# Autodesk Inventor assembly: Ensamble EVA
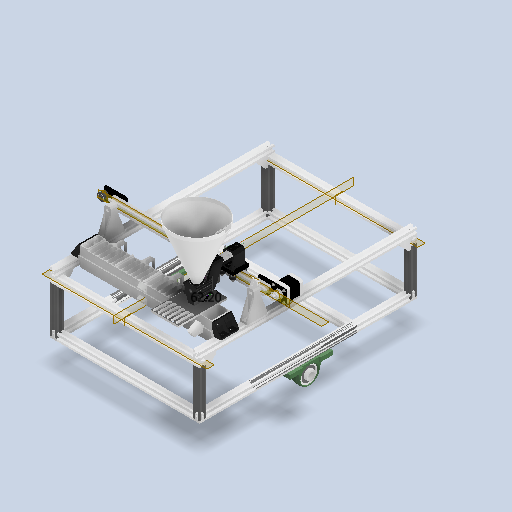
[picture p0: Inventor's stored thumbnail of the model, 512x512]
Saved by Autodesk Inventor 2022 (Build 260153000, 153)
## iProperties
Created: 2021-02-21
Part Number: Ensamble EVA
Document SubType Name: Assembly
Designer: juanp
Author: juanp
## Documents named in this file (12)
- C:\Users\juanp\Desktop\Robocol\EVA\V2 (Antiguo)\Ensamble EVA V2.iam
- C:\Users\juanp\Desktop\Robocol\EVA\Recursos\Actuador Lineal\Actuador Lineal (sin carro).iam
- C:\Users\juanp\Desktop\Robocol\EVA\Recursos\Chasis\Diseño 1.3 (2020)\Ensamble_chasis.iam
- C:\Users\juanp\Desktop\Robocol\EVA\Recursos\Actuador Lineal\Carro deslizante\Carro Deslizante.ipt
- C:\Users\juanp\Desktop\Robocol\EVA\V2 (Antiguo)\Dispensador\Dispensador V2.iam
- C:\Users\juanp\Desktop\Robocol\EVA\V2 (Antiguo)\Cajas\cajas_V2.iam
- C:\Users\juanp\Desktop\Robocol\EVA\V2 (Antiguo)\Acople a chasis\Soporte.ipt
- C:\Users\juanp\Desktop\Robocol\EVA\V2 (Antiguo)\Acople a chasis\Soporte Cajas.ipt
- C:\Users\juanp\Desktop\Robocol\EVA\V2 (Antiguo)\Sostenedor MQ.ipt
- C:\Users\juanp\Desktop\Robocol\EVA\Recursos\Sensores\MQ2\MQ-2.iam
- C:\Users\juanp\Desktop\Robocol\EVA\Recursos\Fin de carrera\Fin de carrera.ipt
- C:\Users\juanp\Desktop\Robocol\EVA\V2 (Antiguo)\Acople a chasis\Soporte ajustado a deflexion - fin de carrera.ipt
## Components (13 placed, 11 different names)
1. Actuador Lineal (sin carro):1 [sub-assembly] — Angle:1, Angle:2, Mate:1, Angle:3, Angle:4, Flush:2, Mate:3, Angle:5, Flush:4, Mate:48, Mate:50, Mate:57
2. Ensamble_chasis:1 [sub-assembly] — Angle:1, Angle:2, Mate:1, Flush:3, Flush:5, Flush:6, Mate:52, Mate:55, Mate:58, Mate:59, Flush:9, Mate:65, Flush:10
3. Carro Deslizante:1 — Angle:3, Angle:4, Flush:2, Mate:3, Mate:42, Mate:43, Mate:44
4. Dispensador V2:1 [sub-assembly] — Mate:42, Mate:43, Mate:44, Mate:46, Mate:60
5. cajas_V2:1 [sub-assembly] — Angle:5, Flush:3, Mate:46, Flush:4, Mate:53, Flush:7, Mate:54, Flush:8, Flush:9
6. Soporte:1 — Flush:5, Mate:48, Mate:57, Mate:58, Flush:11
7. Soporte:2 — Flush:6, Mate:50, Mate:59
8. Soporte Cajas:1 — Mate:52, Mate:53, Flush:7
9. Soporte Cajas:2 — Mate:54, Mate:55, Flush:8
10. Sostenedor MQ:1 — Mate:60, Mate:61, Mate:62, Mate:63
11. MQ-2:1 [sub-assembly] — Mate:61, Mate:62, Mate:63
12. Fin de carrera:1 — Mate:66, Mate:67, Mate:68
13. Soporte ajustado a deflexion - fin de carrera:1 — Mate:65, Flush:10, Flush:11, Mate:66, Mate:67, Mate:68
## Relationships (38: Mate 23, Flush 10, Angle 5)
- Angle:1 (180 deg): Actuador Lineal (sin carro):1 ↔ Ensamble_chasis:1
- Angle:2 (0 deg): Actuador Lineal (sin carro):1 ↔ Ensamble_chasis:1
- Mate:1: Actuador Lineal (sin carro):1 ↔ Ensamble_chasis:1
- Angle:3 (0 deg): Actuador Lineal (sin carro):1 ↔ Carro Deslizante:1
- Angle:4 (180 deg): Actuador Lineal (sin carro):1 ↔ Carro Deslizante:1
- Flush:2: Actuador Lineal (sin carro):1 ↔ Carro Deslizante:1
- Mate:3: Actuador Lineal (sin carro):1 ↔ Carro Deslizante:1
- Mate:42: Carro Deslizante:1 ↔ Dispensador V2:1
- Mate:43: Carro Deslizante:1 ↔ Dispensador V2:1
- Mate:44: Carro Deslizante:1 ↔ Dispensador V2:1
- Angle:5 (180 deg): Actuador Lineal (sin carro):1 ↔ cajas_V2:1
- Flush:3: Ensamble_chasis:1 ↔ cajas_V2:1
- Mate:46 (5.583 mm): Dispensador V2:1 ↔ cajas_V2:1
- Flush:4: Actuador Lineal (sin carro):1 ↔ cajas_V2:1
- Flush:5: Ensamble_chasis:1 ↔ Soporte:1
- Mate:48: Actuador Lineal (sin carro):1 ↔ Soporte:1
- Flush:6: Ensamble_chasis:1 ↔ Soporte:2
- Mate:50: Actuador Lineal (sin carro):1 ↔ Soporte:2
- Mate:52: Ensamble_chasis:1 ↔ Soporte Cajas:1
- Mate:53: cajas_V2:1 ↔ Soporte Cajas:1
- Flush:7: cajas_V2:1 ↔ Soporte Cajas:1
- Mate:54: cajas_V2:1 ↔ Soporte Cajas:2
- Mate:55: Ensamble_chasis:1 ↔ Soporte Cajas:2
- Flush:8: cajas_V2:1 ↔ Soporte Cajas:2
- Mate:57: Actuador Lineal (sin carro):1 ↔ Soporte:1
- Mate:58: Ensamble_chasis:1 ↔ Soporte:1
- Mate:59: Ensamble_chasis:1 ↔ Soporte:2
- Mate:60: Dispensador V2:1 ↔ Sostenedor MQ:1
- Mate:61: Sostenedor MQ:1 ↔ MQ-2:1
- Mate:62: Sostenedor MQ:1 ↔ MQ-2:1
- Mate:63: Sostenedor MQ:1 ↔ MQ-2:1
- Flush:9: Ensamble_chasis:1 ↔ cajas_V2:1
- Mate:65: Ensamble_chasis:1 ↔ Soporte ajustado a deflexion - fin de carrera:1
- Flush:10: Ensamble_chasis:1 ↔ Soporte ajustado a deflexion - fin de carrera:1
- Flush:11: Soporte:1 ↔ Soporte ajustado a deflexion - fin de carrera:1
- Mate:66: Fin de carrera:1 ↔ Soporte ajustado a deflexion - fin de carrera:1
- Mate:67: Fin de carrera:1 ↔ Soporte ajustado a deflexion - fin de carrera:1
- Mate:68: Fin de carrera:1 ↔ Soporte ajustado a deflexion - fin de carrera:1
